# Autodesk Inventor assembly: Box Assembly
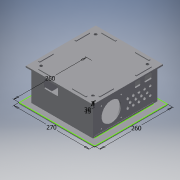
[picture p0: Inventor's stored thumbnail of the model, 180x180]
Saved by Autodesk Inventor 2019 (Build 230136000, 136)
## iProperties
Created: 2019-07-09
Part Number: Box Assembly
Document SubType Name: Assembly
Designer: azriel
Author: azriel
## Documents named in this file (7)
- C:\Users\azriel\Desktop\Box\Box Assembly.iam
- C:\Users\azriel\Desktop\Box\Part Buttom.ipt
- C:\Users\azriel\Desktop\Box\Part Sisi 1.ipt
- C:\Users\azriel\Desktop\Box\Part Sisi 2.ipt
- C:\Users\azriel\Desktop\Box\Part Sisi 3.ipt
- C:\Users\azriel\Desktop\Box\Part Sisi 4.ipt
- C:\Users\azriel\Desktop\Box\Part Upper.ipt
## Components (6 placed, 6 different names)
1. Part Buttom:1 — Mate:1, Mate:2, Mate:3, Mate:4, Mate:5, Mate:6, Mate:10, Mate:11, Mate:12, Mate:18, Mate:19, Mate:20
2. Part Sisi 1:1 — Mate:1, Mate:2, Mate:3
3. Part Sisi 2:1 — Mate:4, Mate:5, Mate:6
4. Part Sisi 3:1 — Mate:18, Mate:19, Mate:20
5. Part Sisi 4:1 — Mate:10, Mate:11, Mate:12, Mate:17
6. Part Upper:1 — Mate:17
## Relationships (13: Mate 13)
- Mate:1: Part Buttom:1 ↔ Part Sisi 1:1
- Mate:2: Part Buttom:1 ↔ Part Sisi 1:1
- Mate:3: Part Buttom:1 ↔ Part Sisi 1:1
- Mate:4: Part Buttom:1 ↔ Part Sisi 2:1
- Mate:5: Part Buttom:1 ↔ Part Sisi 2:1
- Mate:6: Part Buttom:1 ↔ Part Sisi 2:1
- Mate:10: Part Buttom:1 ↔ Part Sisi 4:1
- Mate:11: Part Buttom:1 ↔ Part Sisi 4:1
- Mate:12: Part Buttom:1 ↔ Part Sisi 4:1
- Mate:17: Part Sisi 4:1 ↔ Part Upper:1
- Mate:18: Part Buttom:1 ↔ Part Sisi 3:1
- Mate:19: Part Buttom:1 ↔ Part Sisi 3:1
- Mate:20: Part Buttom:1 ↔ Part Sisi 3:1
